# Autodesk Inventor assembly: Assembly1
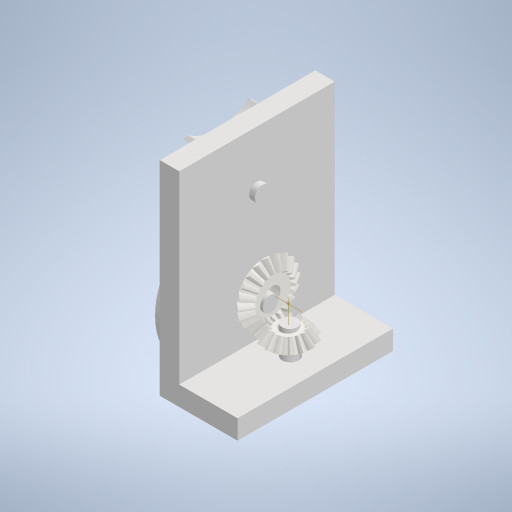
[picture p0: Inventor's stored thumbnail of the model, 512x512]
Saved by Autodesk Inventor 2023 (Build 270158000, 158)
## iProperties
Created: 2023-01-31
Part Number: Assembly1
Document SubType Name: Assembly
Designer: Shishir Gujarey
Author: Shishir Gujarey
## Documents named in this file (7)
- D:\Desktop\Assembly1.iam
- D:\Desktop\Support Plate.ipt
- D:\Desktop\Geneva Driver Wheel.ipt
- D:\Desktop\Geneva Driven Wheel.ipt
- D:\Desktop\Shaft.ipt
- D:\Desktop\Bevel Gears1.iam
- D:\Desktop\Bevel Gears2.iam
## Components (8 placed, 5 different names)
1. Support Plate:1 — Mate:1, Mate:2, Mate:4, Mate:7, Mate:9
2. Geneva Driver Wheel:1 — Mate:1, Mate:2, Mate:3, Mate:8, Rotation:4, Mate:13
3. Geneva Driven Wheel:1 — Mate:3, Mate:4, Mate:5, Mate:6, Mate:14
4. Shaft:1 — Mate:5, Mate:6, Mate:14
5. Shaft:2 — Mate:7, Mate:8, Mate:10, Rotation:3, Rotation:4, Mate:13
6. Shaft:3 — Mate:9, Mate:11, Flush:1, Rotation:2
7. Bevel Gears:1 [sub-assembly] — Mate:10, Mate:12, Rotation:1, Rotation:3
8. Bevel Gears:2 [sub-assembly] — Mate:11, Mate:12, Flush:1, Rotation:1, Rotation:2
## Relationships (19: Mate 14, RelateRotation 4, Flush 1)
- Mate:1: Support Plate:1 ↔ Geneva Driver Wheel:1
- Mate:2: Support Plate:1 ↔ Geneva Driver Wheel:1
- Mate:3: Geneva Driver Wheel:1 ↔ Geneva Driven Wheel:1
- Mate:4: Support Plate:1 ↔ Geneva Driven Wheel:1
- Mate:5: Geneva Driven Wheel:1 ↔ Shaft:1
- Mate:6: Geneva Driven Wheel:1 ↔ Shaft:1
- Mate:7: Support Plate:1 ↔ Shaft:2
- Mate:8: Geneva Driver Wheel:1 ↔ Shaft:2
- Mate:9: Support Plate:1 ↔ Shaft:3
- Mate:10: Shaft:2 ↔ Bevel Gears:1
- Mate:11: Shaft:3 ↔ Bevel Gears:2
- Mate:12: Bevel Gears:1 ↔ Bevel Gears:2
- Flush:1: Shaft:3 ↔ Bevel Gears:2
- Rotation:1 [RelateRotation] (1.3333 ul): Bevel Gears:1 ↔ Bevel Gears:2
- Rotation:2 [RelateRotation] (1 ul): Shaft:3 ↔ Bevel Gears:2
- Rotation:3 [RelateRotation] (1 ul): Shaft:2 ↔ Bevel Gears:1
- Rotation:4 [RelateRotation] (1 ul): Geneva Driver Wheel:1 ↔ Shaft:2
- Mate:13: Geneva Driver Wheel:1 ↔ Shaft:2
- Mate:14: Geneva Driven Wheel:1 ↔ Shaft:1
